# Autodesk Inventor assembly: left wheel_MIR
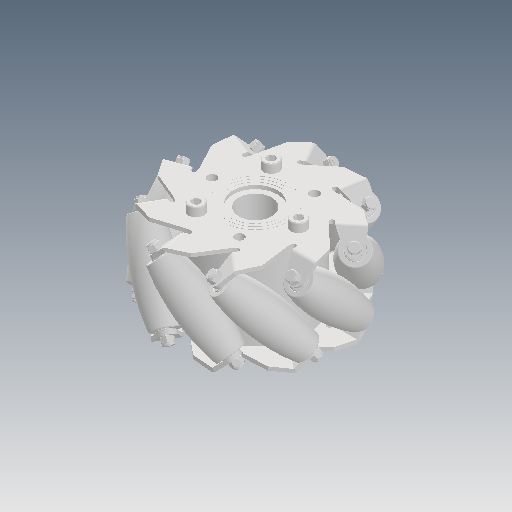
[picture p0: Inventor's stored thumbnail of the model, 512x512]
Saved by Autodesk Inventor 2020 (Build 240168000, 168)
## iProperties
Created: 2019-09-27
Part Number: left wheel_MIR
Document SubType Name: Assembly
Designer: ball
Author: ball
## Documents named in this file (4)
- C:\FTC\FTC8863CAD\2019 Robot\Mecanum Drive Train\left wheel_MIR.iam
- C:\FTC\FTC8863CAD\StepLibraries\Screws\M5 x 55 SOCKET HEAD CAP SCREW_MIR.ipt
- C:\FTC\FTC8863CAD\StepLibraries\Nuts\M5 NYLON-INSERT LOCKNUT_MIR.ipt
- C:\FTC\FTC8863CAD\Nexus-Wheels-STP\100mm Aluminum Mecanum wheels_MIR.ipt
## Components (7 placed, 3 different names)
1. M5 x 55 SOCKET HEAD CAP SCREW_MIR:1 — Mate:11, Mate:2, Mate:1
2. M5 NYLON-INSERT LOCKNUT_MIR:1 — Mate:7, Mate:12
3. 100mm Aluminum Mecanum wheels_MIR:1 — Mate:7, Mate:8, Mate:9, Mate:2, Mate:1, Mate:5, Mate:4, Mate:6, Mate:3
4. M5 x 55 SOCKET HEAD CAP SCREW_MIR:2 — Mate:12, Mate:5, Mate:4
5. M5 x 55 SOCKET HEAD CAP SCREW_MIR:3 — Mate:10, Mate:6, Mate:3
6. M5 NYLON-INSERT LOCKNUT_MIR:2 — Mate:8, Mate:10
7. M5 NYLON-INSERT LOCKNUT_MIR:3 — Mate:9, Mate:11
## Relationships (12: Mate 12)
- Mate:7: M5 NYLON-INSERT LOCKNUT_MIR:1 ↔ 100mm Aluminum Mecanum wheels_MIR:1
- Mate:8: 100mm Aluminum Mecanum wheels_MIR:1 ↔ M5 NYLON-INSERT LOCKNUT_MIR:2
- Mate:9: 100mm Aluminum Mecanum wheels_MIR:1 ↔ M5 NYLON-INSERT LOCKNUT_MIR:3
- Mate:11: M5 x 55 SOCKET HEAD CAP SCREW_MIR:1 ↔ M5 NYLON-INSERT LOCKNUT_MIR:3
- Mate:2: M5 x 55 SOCKET HEAD CAP SCREW_MIR:1 ↔ 100mm Aluminum Mecanum wheels_MIR:1
- Mate:1: M5 x 55 SOCKET HEAD CAP SCREW_MIR:1 ↔ 100mm Aluminum Mecanum wheels_MIR:1
- Mate:12: M5 NYLON-INSERT LOCKNUT_MIR:1 ↔ M5 x 55 SOCKET HEAD CAP SCREW_MIR:2
- Mate:5: 100mm Aluminum Mecanum wheels_MIR:1 ↔ M5 x 55 SOCKET HEAD CAP SCREW_MIR:2
- Mate:4: 100mm Aluminum Mecanum wheels_MIR:1 ↔ M5 x 55 SOCKET HEAD CAP SCREW_MIR:2
- Mate:10: M5 x 55 SOCKET HEAD CAP SCREW_MIR:3 ↔ M5 NYLON-INSERT LOCKNUT_MIR:2
- Mate:6: 100mm Aluminum Mecanum wheels_MIR:1 ↔ M5 x 55 SOCKET HEAD CAP SCREW_MIR:3
- Mate:3: 100mm Aluminum Mecanum wheels_MIR:1 ↔ M5 x 55 SOCKET HEAD CAP SCREW_MIR:3
